# Autodesk Inventor assembly: A_aluminium
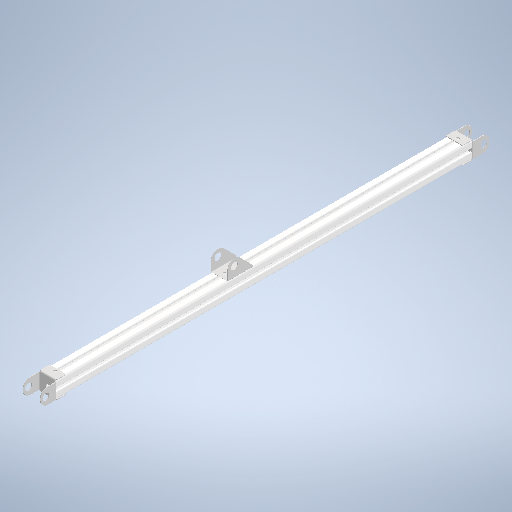
[picture p0: Inventor's stored thumbnail of the model, 512x512]
Saved by Autodesk Inventor 2025.2 (Build 292293000, 293)
## iProperties
Created: 2025-04-29
Part Number: A_aluminium
Document SubType Name: Assembly
Designer: Caspe
Author: Caspe
## Documents named in this file (4)
- C:\Users\Caspe\Documents\Semester 8\Project\Anomaly_Detection\Mechanical_Project\Inventor_project\A_aluminium.iam
- C:\Users\Caspe\Documents\Semester 8\Project\Anomaly_Detection\Mechanical_Project\Inventor_project\0_0_026_03-1000-Aluflex\0_0_026_03-1000-Aluflex\0_0_026_03-1000-Aluflex.ipt
- C:\Users\Caspe\Documents\Semester 8\Project\Anomaly_Detection\Mechanical_Project\Inventor_project\profile_mount-1.ipt
- C:\Users\Caspe\Documents\Semester 8\Project\Anomaly_Detection\Mechanical_Project\Inventor_project\profile_mount-2.ipt
## Components (4 placed, 3 different names)
1. 0_0_026_03-1000-Aluflex:1 — Mate:1, Flush:1, Insert:1, Mate:2, Insert:2, Mate:3
2. profile_mount-1:1 — Mate:1, Flush:1
3. profile_mount-2:1 — Insert:1, Mate:2
4. profile_mount-2:2 — Insert:2, Mate:3
## Relationships (6: Mate 3, Insert 2, Flush 1)
- Mate:1: 0_0_026_03-1000-Aluflex:1 ↔ profile_mount-1:1
- Flush:1: 0_0_026_03-1000-Aluflex:1 ↔ profile_mount-1:1
- Insert:1: 0_0_026_03-1000-Aluflex:1 ↔ profile_mount-2:1
- Mate:2: 0_0_026_03-1000-Aluflex:1 ↔ profile_mount-2:1
- Insert:2: 0_0_026_03-1000-Aluflex:1 ↔ profile_mount-2:2
- Mate:3: 0_0_026_03-1000-Aluflex:1 ↔ profile_mount-2:2
